# Autodesk Inventor assembly: Estructura matriz centelladora
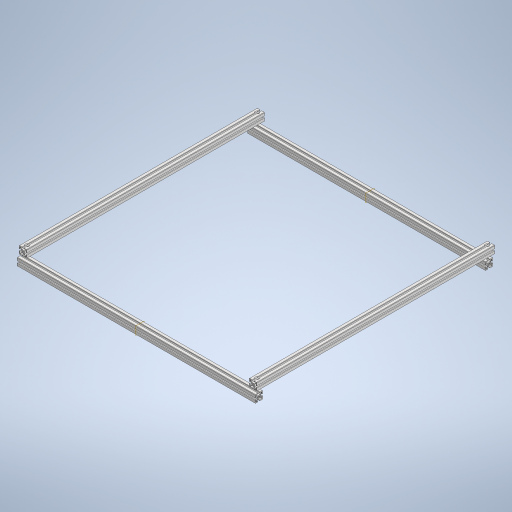
[picture p0: Inventor's stored thumbnail of the model, 512x512]
Saved by Autodesk Inventor 2024.2 (Build 282272000, 272)
## iProperties
Created: 2024-08-23
Part Number: Estructura matriz centelladora
Document SubType Name: Assembly
Designer: ja.restrepo1
Author: ja.restrepo1
## Documents named in this file (4)
- I:\MICROMECANICA\ALTAS ENERGIAS\Deteccion de Muones\Detectores\Detectores centelladores\Partes Detectores centelladores\PARTES DC\Perfileria 20x20 DC\Estructura matriz centelladora.iam
- I:\MICROMECANICA\ALTAS ENERGIAS\Deteccion de Muones\Detectores\Detectores centelladores\Partes Detectores centelladores\PARTES DC\Perfileria 20x20 DC\Perfil 20X20 T.ipt
- I:\MICROMECANICA\ALTAS ENERGIAS\Deteccion de Muones\Detectores\Detectores centelladores\Partes Detectores centelladores\PARTES DC\Perfileria 20x20 DC\Perfil 20X20 T\Perfil 20X20 T-620BCAM5.ipt
- I:\MICROMECANICA\ALTAS ENERGIAS\Deteccion de Muones\Detectores\Detectores centelladores\Partes Detectores centelladores\PARTES DC\Perfileria 20x20 DC\Perfil 20X20 T\Perfil 20X20 T-620M5.ipt
## Components (4 placed, 2 different names)
1. Perfil 20X20 T-620BCAM5:1 — Flush:2, Mate:1, Flush:3, Mate:2, Flush:4
2. Perfil 20X20 T-620BCAM5:2 — Flush:1, Mate:1, Flush:3, Flush:8, Flush:9, Mate:3
3. Perfil 20X20 T-620M5:3 — Flush:6, Flush:7, Flush:8, Mate:3
4. Perfil 20X20 T-620M5:4 — Flush:5, Flush:7, Flush:9
## Relationships (12: Flush 9, Mate 3)
- Flush:1: Perfil 20X20 T-620BCAM5:2
- Flush:2: Perfil 20X20 T-620BCAM5:1
- Mate:1 (580 mm): Perfil 20X20 T-620BCAM5:1 ↔ Perfil 20X20 T-620BCAM5:2
- Flush:3: Perfil 20X20 T-620BCAM5:1 ↔ Perfil 20X20 T-620BCAM5:2
- Mate:2 (5 mm): Perfil 20X20 T-620BCAM5:1
- Flush:4 (295 mm): Perfil 20X20 T-620BCAM5:1
- Flush:5: Perfil 20X20 T-620M5:4
- Flush:6: Perfil 20X20 T-620M5:3
- Flush:7: Perfil 20X20 T-620M5:3 ↔ Perfil 20X20 T-620M5:4
- Flush:8: Perfil 20X20 T-620BCAM5:2 ↔ Perfil 20X20 T-620M5:3
- Flush:9: Perfil 20X20 T-620BCAM5:2 ↔ Perfil 20X20 T-620M5:4
- Mate:3 (10 mm): Perfil 20X20 T-620BCAM5:2 ↔ Perfil 20X20 T-620M5:3
